# Autodesk Inventor assembly: Potential gripper
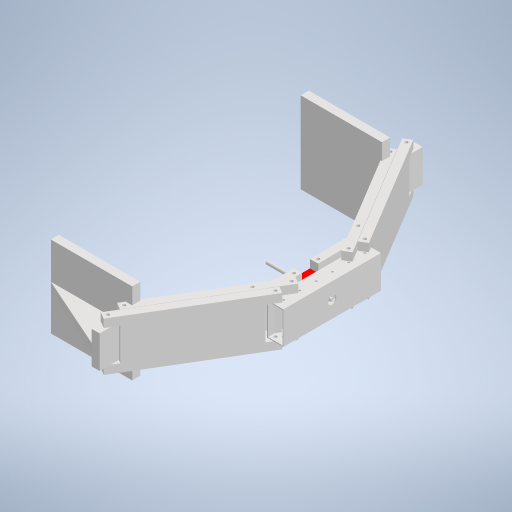
[picture p0: Inventor's stored thumbnail of the model, 512x512]
Saved by Autodesk Inventor 2023 (Build 270158000, 158)
## iProperties
Created: 2023-01-25
Part Number: Potential gripper
Document SubType Name: Assembly
Designer: Gabriel - T3 CAD
Author: Gabriel - T3 CAD
## Documents named in this file (8)
- C:\Users\Gabriel - T3 CAD\Documents\GitHub\t3-CAD\T3-CAD\Current Season CAD\Swerve-DriveTrain-V2.1 (LongBot)\Potential new gripper\Potential gripper.iam
- C:\Users\Gabriel - T3 CAD\Documents\GitHub\t3-CAD\T3-CAD\Current Season CAD\Swerve-DriveTrain-V2.1 (LongBot)\Potential new gripper\VersaFrame (arm base).ipt
- C:\Users\Gabriel - T3 CAD\Documents\GitHub\t3-CAD\T3-CAD\Current Season CAD\Swerve-DriveTrain-V2.1 (LongBot)\Potential new gripper\outer swing.ipt
- C:\Users\Gabriel - T3 CAD\Documents\GitHub\t3-CAD\T3-CAD\Current Season CAD\Swerve-DriveTrain-V2.1 (LongBot)\Potential new gripper\inner swing.ipt
- C:\Users\Gabriel - T3 CAD\Documents\GitHub\t3-CAD\T3-CAD\Current Season CAD\Swerve-DriveTrain-V2.1 (LongBot)\Potential new gripper\swing pusher.ipt
- C:\Users\Gabriel - T3 CAD\Documents\GitHub\t3-CAD\T3-CAD\Current Season CAD\Swerve-DriveTrain-V2.1 (LongBot)\Potential new gripper\piston connection.ipt
- C:\Users\Gabriel - T3 CAD\Documents\GitHub\t3-CAD\T3-CAD\Current Season CAD\Swerve-DriveTrain-V2.1 (LongBot)\Potential new gripper\Finger.ipt
- C:\Users\Gabriel - T3 CAD\Documents\GitHub\t3-CAD\T3-CAD\Current Season CAD\Swerve-DriveTrain-V2.1 (LongBot)\Potential new gripper\piston stand in.ipt
## Components (11 placed, 7 different names)
1. VersaFrame (arm base):1 — Mate:1, Mate:2, Mate:3, Mate:4, Mate:5, Mate:6, Mate:7, Mate:8, Rigid:1
2. outer swing:1 — Mate:1, Mate:2, Mate:20, Mate:21
3. outer swing:2 — Mate:3, Mate:4, Mate:22, Mate:23
4. inner swing:1 — Mate:7, Mate:8, Mate:16, Mate:17, Mate:24, Mate:25
5. inner swing:2 — Mate:5, Mate:6, Mate:9, Mate:12, Mate:18, Mate:19
6. swing pusher:1 — Mate:9, Mate:12, Mate:15
7. swing pusher:2 — Mate:13, Mate:14, Mate:16, Mate:17
8. piston connection:1 — Mate:13, Mate:14, Mate:15, Cylindrical:1
9. Finger:1 — Mate:18, Mate:19, Mate:20, Mate:21
10. Finger:2 — Mate:22, Mate:23, Mate:24, Mate:25
11. piston stand in:1 — Rigid:1, Cylindrical:1
## Relationships (25: Mate 23, WeldJoint 1, CylindricalJoint 1)
- Mate:1: VersaFrame (arm base):1 ↔ outer swing:1
- Mate:2: VersaFrame (arm base):1 ↔ outer swing:1
- Mate:3: VersaFrame (arm base):1 ↔ outer swing:2
- Mate:4: VersaFrame (arm base):1 ↔ outer swing:2
- Mate:5: VersaFrame (arm base):1 ↔ inner swing:2
- Mate:6: VersaFrame (arm base):1 ↔ inner swing:2
- Mate:7: VersaFrame (arm base):1 ↔ inner swing:1
- Mate:8: VersaFrame (arm base):1 ↔ inner swing:1
- Mate:9: inner swing:2 ↔ swing pusher:1
- Mate:12: inner swing:2 ↔ swing pusher:1
- Mate:13: swing pusher:2 ↔ piston connection:1
- Mate:14: swing pusher:2 ↔ piston connection:1
- Mate:15: swing pusher:1 ↔ piston connection:1
- Mate:16: inner swing:1 ↔ swing pusher:2
- Mate:17: inner swing:1 ↔ swing pusher:2
- Mate:18: inner swing:2 ↔ Finger:1
- Mate:19: inner swing:2 ↔ Finger:1
- Mate:20: outer swing:1 ↔ Finger:1
- Mate:21: outer swing:1 ↔ Finger:1
- Mate:22: outer swing:2 ↔ Finger:2
- Mate:23: outer swing:2 ↔ Finger:2
- Mate:24: inner swing:1 ↔ Finger:2
- Mate:25: inner swing:1 ↔ Finger:2
- Rigid:1 [WeldJoint]: VersaFrame (arm base):1 ↔ piston stand in:1
- Cylindrical:1: piston connection:1 ↔ piston stand in:1
